# Autodesk Inventor assembly: Print 2
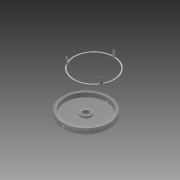
[picture p0: Inventor's stored thumbnail of the model, 180x180]
Saved by Autodesk Inventor 2014 (Build 180170000, 170)
## iProperties
Created: 2015-03-30
Part Number: Print 2
Document SubType Name: Assembly
Designer: MSI
Author: MSI
## Documents named in this file (3)
- C:\Users\MSI\Dropbox\Ingenieursproject\inventor\Print 2.iam
- C:\Users\MSI\Dropbox\Ingenieursproject\inventor\Hallhouder.ipt
- C:\Users\MSI\Dropbox\Ingenieursproject\inventor\rotor.ipt
## Components (2 placed, 2 different names)
1. Hallhouder:1 — Mate:2
2. rotor:1 — Mate:1
## Relationships (3: Mate 2, Flush 1)
- Flush:1
- Mate:1: rotor:1
- Mate:2: Hallhouder:1
